# Autodesk Inventor assembly: HeroeEnsamblado
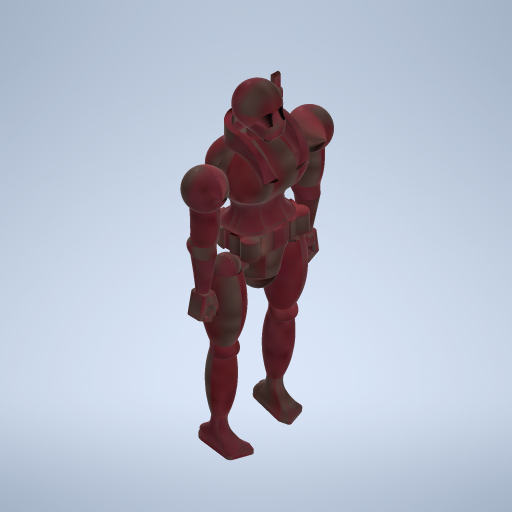
[picture p0: Inventor's stored thumbnail of the model, 512x512]
Saved by Autodesk Inventor 2024.3 (Build 283343000, 343)
## iProperties
Created: 2025-01-26
Part Number: HeroeEnsamblado
Document SubType Name: Assembly
Designer: USUARIO
Author: USUARIO
## Documents named in this file (7)
- D:\USUARIO\Documents\Universidad Andres\2024-2\apm\HeroeEnsamblado.iam
- D:\USUARIO\Documents\Universidad Andres\2024-2\apm\H-torso.ipt
- D:\USUARIO\Documents\Universidad Andres\2024-2\apm\H_piernader.ipt
- D:\USUARIO\Documents\Universidad Andres\2024-2\apm\H_piernaIzq.ipt
- D:\USUARIO\Documents\Universidad Andres\2024-2\apm\H-brazoIzq.ipt
- D:\USUARIO\Documents\Universidad Andres\2024-2\apm\H-brazoDer.ipt
- D:\USUARIO\Documents\Universidad Andres\2024-2\apm\H-cabeza.ipt
## Components (6 placed, 6 different names)
1. H-torso:1 — Mate:1, Mate:2, Mate:3, Mate:4, Mate:5, Mate:6, Mate:7, Mate:8, Mate:9, Mate:10
2. H_piernader:1 — Mate:5, Mate:6
3. H_piernaIzq:1 — Mate:7, Mate:8
4. H-brazoIzq:1 — Mate:3, Mate:4
5. H-brazoDer:1 — Mate:1, Mate:2
6. H-cabeza:1 — Mate:9, Mate:10
## Relationships (10: Mate 10)
- Mate:1: H-torso:1 ↔ H-brazoDer:1
- Mate:2 (3 mm): H-torso:1 ↔ H-brazoDer:1
- Mate:3: H-torso:1 ↔ H-brazoIzq:1
- Mate:4 (3 mm): H-torso:1 ↔ H-brazoIzq:1
- Mate:5: H-torso:1 ↔ H_piernader:1
- Mate:6 (-8 mm): H-torso:1 ↔ H_piernader:1
- Mate:7: H-torso:1 ↔ H_piernaIzq:1
- Mate:8 (-8 mm): H-torso:1 ↔ H_piernaIzq:1
- Mate:9: H-torso:1 ↔ H-cabeza:1
- Mate:10 (3 mm): H-torso:1 ↔ H-cabeza:1
